# Autodesk Inventor assembly: BASE1
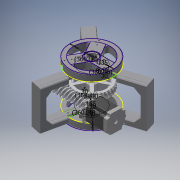
[picture p0: Inventor's stored thumbnail of the model, 180x180]
Saved by Autodesk Inventor 2017 (Build 210142000, 142)
## iProperties
Created: 2016-12-27
Part Number: BASE1
Document SubType Name: Assembly
Designer: Samanth
Author: Samanth
## Documents named in this file (5)
- C:\Users\Samanth\Desktop\Purdue Files\Robot\BASE1.iam
- C:\Users\Samanth\Desktop\Purdue Files\Robot\Base1.ipt
- C:\Users\Samanth\Desktop\Purdue Files\Robot\doubleHelix\Design Accelerator\Worm Gears1.iam
- C:\Users\Samanth\Desktop\Purdue Files\Robot\Stepper motor NEMA 23HS7430.ipt
- C:\Users\Samanth\Desktop\Purdue Files\Robot\BaseSupport.ipt
## Components (7 placed, 4 different names)
1. Base1:1 — Mate:1, Mate:2, Mate:3
2. Base1:2 — Mate:1, Mate:2, Mate:4, Mate:7, Mate:8, Mate:9, Mate:10, Mate:11, Mate:12, Mate:13, Mate:14, Mate:15
3. Worm Gears:1 [sub-assembly] — Mate:3, Mate:4, Mate:5, Mate:6
4. Stepper motor NEMA 23HS7430:1 — Mate:5, Mate:6
5. BaseSupport:1 — Mate:7, Mate:8, Mate:9
6. BaseSupport:2 — Mate:10, Mate:11, Mate:12
7. BaseSupport:3 — Mate:13, Mate:14, Mate:15
## Relationships (15: Mate 15)
- Mate:1: Base1:1 ↔ Base1:2
- Mate:2 (110 mm): Base1:1 ↔ Base1:2
- Mate:3: Base1:1 ↔ Worm Gears:1
- Mate:4 (45 mm): Base1:2 ↔ Worm Gears:1
- Mate:5: Worm Gears:1 ↔ Stepper motor NEMA 23HS7430:1
- Mate:6 (5 mm): Worm Gears:1 ↔ Stepper motor NEMA 23HS7430:1
- Mate:7: Base1:2 ↔ BaseSupport:1
- Mate:8: Base1:2 ↔ BaseSupport:1
- Mate:9: Base1:2 ↔ BaseSupport:1
- Mate:10: Base1:2 ↔ BaseSupport:2
- Mate:11: Base1:2 ↔ BaseSupport:2
- Mate:12: Base1:2 ↔ BaseSupport:2
- Mate:13: Base1:2 ↔ BaseSupport:3
- Mate:14: Base1:2 ↔ BaseSupport:3
- Mate:15: Base1:2 ↔ BaseSupport:3
